# Autodesk Inventor assembly: BackUpperLink
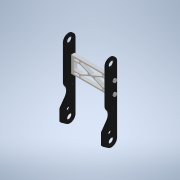
[picture p0: Inventor's stored thumbnail of the model, 180x180]
Saved by Autodesk Inventor 2022.3 (Build 263350000, 350)
## iProperties
Created: 2022-06-15
Part Number: BackUpperLink
Document SubType Name: Assembly
Designer: Masato Kubotera
Author: Masato Kubotera
## Documents named in this file (4)
- C:\Users\Masato\Desktop\SUSTAINA-OP\LowerBody\Link\BackUpperLink.iam
- C:\Users\Masato\Desktop\SUSTAINA-OP\LowerBody\Link\BackLink_diagonal.ipt
- C:\Users\Masato\Desktop\SUSTAINA-OP\LowerBody\Link\BackLink_frame.ipt
- C:\Users\Masato\Desktop\SUSTAINA-OP\ReadyMade\Screw\M3-6.ipt
## Components (7 placed, 3 different names)
1. BackLink_diagonal:1 — フラッシュ:1, フラッシュ:2, フラッシュ:3, 挿入:1, 挿入:2, 挿入:3, 挿入:4
2. BackLink_frame:1 — 挿入:1, 挿入:2, 挿入:5, 挿入:6
3. BackLink_frame:2 — 挿入:3, 挿入:4, 挿入:7, 挿入:8
4. M3-6:1 — 挿入:5
5. M3-6:2 — 挿入:6
6. M3-6:3 — 挿入:7
7. M3-6:4 — 挿入:8
## Relationships (11: Insert 8, Flush 3)
- フラッシュ:1 [Flush]: BackLink_diagonal:1
- フラッシュ:2 [Flush]: BackLink_diagonal:1
- フラッシュ:3 [Flush]: BackLink_diagonal:1
- 挿入:1 [Insert]: BackLink_diagonal:1 ↔ BackLink_frame:1
- 挿入:2 [Insert]: BackLink_diagonal:1 ↔ BackLink_frame:1
- 挿入:3 [Insert]: BackLink_diagonal:1 ↔ BackLink_frame:2
- 挿入:4 [Insert]: BackLink_diagonal:1 ↔ BackLink_frame:2
- 挿入:5 [Insert]: BackLink_frame:1 ↔ M3-6:1
- 挿入:6 [Insert]: BackLink_frame:1 ↔ M3-6:2
- 挿入:7 [Insert]: BackLink_frame:2 ↔ M3-6:3
- 挿入:8 [Insert]: BackLink_frame:2 ↔ M3-6:4
